# Autodesk Inventor assembly: Assembly4
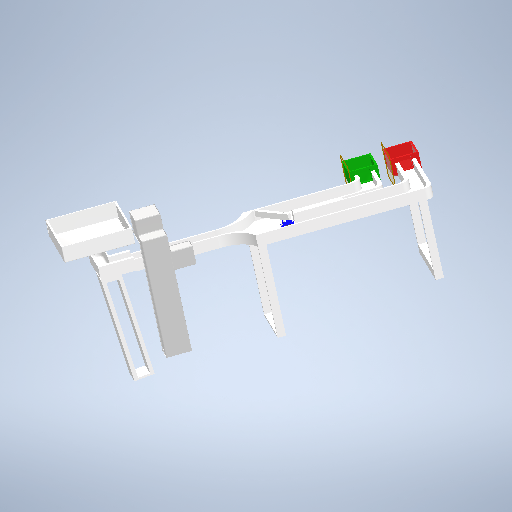
[picture p0: Inventor's stored thumbnail of the model, 512x512]
Saved by Autodesk Inventor 2025.3 (Build 293356000, 356)
## iProperties
Created: 2026-04-16
Part Number: Assembly4
Document SubType Name: Assembly
Designer: tasab
Sending System: Autodesk Inventor 2025
Preprocessor: ST-DEVELOPER v20
Title: Assembly4.stp
Author: tasab
## Documents named in this file (17)
- C:\Users\logys\OneDrive\Desktop\ASU\Spring 2026\Basics of mechatronics\project\Assembly4 sorting.iam
- C:\Users\logys\OneDrive\Desktop\ASU\Spring 2026\Basics of mechatronics\project\sorting lines.ipt
- C:\Users\logys\OneDrive\Desktop\ASU\Spring 2026\Basics of mechatronics\project\servo 1 assembly.iam
- C:\Users\logys\OneDrive\Desktop\ASU\Spring 2026\Basics of mechatronics\project\Part1 svo hand.ipt
- C:\Users\logys\OneDrive\Desktop\ASU\Spring 2026\Basics of mechatronics\project\Part2 colo sns.ipt
- C:\Users\logys\OneDrive\Desktop\ASU\Spring 2026\Basics of mechatronics\project\Part42.ipt
- C:\Users\logys\OneDrive\Desktop\ASU\Spring 2026\Basics of mechatronics\project\TCS3200 Color Sensor Module\TCS3200 Color Sensor Module\TCS3200 Color Sensor Module.ipt
- C:\Users\logys\OneDrive\Desktop\ASU\Spring 2026\Basics of mechatronics\project\Part48.ipt
- C:\Users\logys\OneDrive\Desktop\ASU\Spring 2026\Basics of mechatronics\project\Part1==.ipt
- C:\Users\logys\OneDrive\Desktop\ASU\Spring 2026\Basics of mechatronics\project\catapult assembly\catapult assembly\[4145] TowerPro SG90 Mini Servo-SunRobotics_in-Pt5_BS EN ISO 7045 - M2 x 8 - Z - 8S.ipt
- C:\Users\logys\OneDrive\Desktop\ASU\Spring 2026\Basics of mechatronics\project\sorting track2.ipt
- C:\Users\logys\OneDrive\Desktop\ASU\Spring 2026\Basics of mechatronics\project\sorting track1.ipt
- C:\Users\logys\OneDrive\Desktop\ASU\Spring 2026\Basics of mechatronics\project\sorting box.ipt
- C:\Users\logys\OneDrive\Desktop\ASU\Spring 2026\Machine construction\Project\Assem1\color sensor -servo .ipt
- C:\Users\logys\OneDrive\Desktop\ASU\Spring 2026\Basics of mechatronics\project\cone final.ipt
- C:\Users\logys\OneDrive\Desktop\ASU\Spring 2026\Basics of mechatronics\project\cone base.ipt
- C:\Users\logys\OneDrive\Desktop\ASU\Spring 2026\Basics of mechatronics\project\support1.ipt
## Components (19 placed, 16 different names)
1. sorting lines:1 — Mate:8, Mate:12, Mate:13, Mate:14, Mate:15, Mate:16, Mate:17, Mate:18, Mate:19, Mate:20, Mate:21, Mate:22, Mate:30, Mate:31, Mate:36, Mate:39, Mate:40
2. servo 1 assembly:1 [sub-assembly] — Insert:1, Mate:12, Mate:13, Mate:14, Mate:15
3. servo 1 assembly:2 [sub-assembly] — Insert:2, Mate:8, Mate:16
4. Part1==:1 — Mate:2, Mate:3
5. Part1 svo hand:1 — Insert:1, Mate:2, Mate:3
6. Part2 colo sns:1 — Mate:27, Mate:28, Mate:29, Mate:32, Mate:33, Mate:34, Mate:35, Mate:37, Mate:38
7. Part42:1 — Mate:27, Mate:29, Mate:30
8. Part42:2 — Mate:28, Mate:31, Mate:32, Mate:33, Mate:36
9. T:1 — Mate:34, Mate:35
10. Part48:1 — Insert:2, Mate:9, Mate:10, Mate:17, Mate:18
11. [4145] TowerPro SG90 Mini Servo-SunRobotics_in-Pt5_BS EN ISO 7045 - M2 x 8 - Z - 8S:1 — Mate:9, Mate:10
12. sorting track2:1 — Mate:19, Mate:20, Mate:23, Mate:24
13. sorting track1:1 — Mate:21, Mate:22, Mate:25, Mate:26
14. sorting box:1 — Mate:23, Mate:24
15. sorting box:2 — Mate:25, Mate:26
16. color sensor -servo :1 — Mate:37, Mate:38
17. cone final:1 — Flush:1, Mate:42, Mate:43
18. cone base:1 — Mate:39, Mate:40, Flush:1, Mate:42, Mate:43, Mate:44, Mate:45
19. support1:1 — Mate:44, Mate:45
## Relationships (41: Mate 38, Insert 2, Flush 1)
- Insert:1: servo 1 assembly:1 ↔ Part1 svo hand:1
- Mate:2: Part1==:1 ↔ Part1 svo hand:1
- Mate:3: Part1==:1 ↔ Part1 svo hand:1
- Insert:2: servo 1 assembly:2 ↔ Part48:1
- Mate:8: sorting lines:1 ↔ servo 1 assembly:2
- Mate:9: Part48:1 ↔ [4145] TowerPro SG90 Mini Servo-SunRobotics_in-Pt5_BS EN ISO 7045 - M2 x 8 - Z - 8S:1
- Mate:10: Part48:1 ↔ [4145] TowerPro SG90 Mini Servo-SunRobotics_in-Pt5_BS EN ISO 7045 - M2 x 8 - Z - 8S:1
- Mate:12: sorting lines:1 ↔ servo 1 assembly:1
- Mate:13: sorting lines:1 ↔ servo 1 assembly:1
- Mate:14: sorting lines:1 ↔ servo 1 assembly:1
- Mate:15: sorting lines:1 ↔ servo 1 assembly:1
- Mate:16: sorting lines:1 ↔ servo 1 assembly:2
- Mate:17: sorting lines:1 ↔ Part48:1
- Mate:18: sorting lines:1 ↔ Part48:1
- Mate:19: sorting lines:1 ↔ sorting track2:1
- Mate:20: sorting lines:1 ↔ sorting track2:1
- Mate:21: sorting lines:1 ↔ sorting track1:1
- Mate:22: sorting lines:1 ↔ sorting track1:1
- Mate:23: sorting track2:1 ↔ sorting box:1
- Mate:24: sorting track2:1 ↔ sorting box:1
- Mate:25: sorting track1:1 ↔ sorting box:2
- Mate:26: sorting track1:1 ↔ sorting box:2
- Mate:27: Part2 colo sns:1 ↔ Part42:1
- Mate:28: Part2 colo sns:1 ↔ Part42:2
- Mate:29: Part2 colo sns:1 ↔ Part42:1
- Mate:30: sorting lines:1 ↔ Part42:1
- Mate:31: sorting lines:1 ↔ Part42:2
- Mate:32: Part2 colo sns:1 ↔ Part42:2
- Mate:33: Part2 colo sns:1 ↔ Part42:2
- Mate:34: Part2 colo sns:1 ↔ T:1
- Mate:35: Part2 colo sns:1 ↔ T:1
- Mate:36 (30 mm): sorting lines:1 ↔ Part42:2
- Mate:37: Part2 colo sns:1 ↔ color sensor -servo :1
- Mate:38: Part2 colo sns:1 ↔ color sensor -servo :1
- Mate:39: sorting lines:1 ↔ cone base:1
- Mate:40: sorting lines:1 ↔ cone base:1
- Flush:1: cone final:1 ↔ cone base:1
- Mate:42: cone final:1 ↔ cone base:1
- Mate:43: cone final:1 ↔ cone base:1
- Mate:44: cone base:1 ↔ support1:1
- Mate:45: cone base:1 ↔ support1:1
